# Autodesk Inventor assembly: Ens. Manija
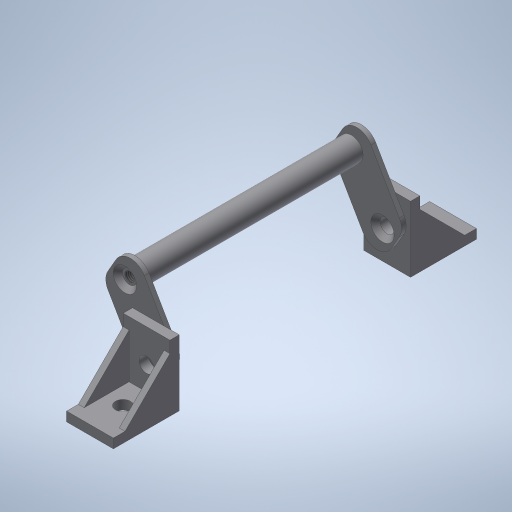
[picture p0: Inventor's stored thumbnail of the model, 512x512]
Saved by Autodesk Inventor 2024.2 (Build 282272000, 272)
## iProperties
Created: 2024-11-25
Part Number: Ens. Manija
Material: Genérico
Document SubType Name: Assembly
Designer: jd.castellanosq
Author: jd.castellanosq
## Documents named in this file (5)
- I:\MICROMECANICA\ALTAS ENERGIAS\Deteccion de Muones\Detectores centelladores\Partes Detectores centelladores\SSE Manija\SSE. Manija.iam
- I:\MICROMECANICA\ALTAS ENERGIAS\Deteccion de Muones\Detectores centelladores\Partes Detectores centelladores\SSE Manija\Lamina.ipt
- I:\MICROMECANICA\ALTAS ENERGIAS\Deteccion de Muones\Detectores centelladores\Partes Detectores centelladores\SSE Manija\eje.ipt
- I:\MICROMECANICA\ALTAS ENERGIAS\Deteccion de Muones\Detectores centelladores\Partes Detectores centelladores\SSE Manija\Escuadra DC.ipt
- I:\MICROMECANICA\ALTAS ENERGIAS\Deteccion de Muones\Detectores centelladores\Partes Detectores centelladores\SSE Manija\Lamina\Lamina Manija.ipt
## Components (5 placed, 3 different names)
1. eje:1 — Flush:1, Flush:2, Flush:3, Mate:1, Mate:2, Mate:3, Mate:7, Mate:9
2. Escuadra DC:1 — Flush:4, Mate:5, Mate:8
3. Escuadra DC:2 — Flush:4, Mate:4, Mate:6
4. Lamina Manija:1 — Mate:2, Mate:5, Mate:8, Mate:9
5. Lamina Manija:2 — Mate:3, Mate:4, Mate:6, Mate:7
## Relationships (13: Mate 9, Flush 4)
- Flush:1: eje:1
- Flush:2: eje:1
- Flush:3: eje:1
- Mate:1: eje:1
- Flush:4: Escuadra DC:1 ↔ Escuadra DC:2
- Mate:2: eje:1 ↔ Lamina Manija:1
- Mate:3: eje:1 ↔ Lamina Manija:2
- Mate:4: Escuadra DC:2 ↔ Lamina Manija:2
- Mate:5: Escuadra DC:1 ↔ Lamina Manija:1
- Mate:6: Escuadra DC:2 ↔ Lamina Manija:2
- Mate:7: eje:1 ↔ Lamina Manija:2
- Mate:8: Escuadra DC:1 ↔ Lamina Manija:1
- Mate:9: eje:1 ↔ Lamina Manija:1
